# Autodesk Inventor assembly: V1
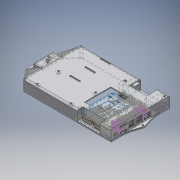
[picture p0: Inventor's stored thumbnail of the model, 180x180]
Saved by Autodesk Inventor 2019 (Build 230136000, 136)
## iProperties
Created: 2020-08-26
Part Number: V1
Document SubType Name: Assembly
Designer: infinity
Author: infinity
## Documents named in this file (4)
- C:\Users\infinity\Documents\GitHub\barc_hardware\Enclosure\XAVIER\V_2\V2.iam
- C:\Users\infinity\Documents\GitHub\barc_hardware\Enclosure\XAVIER\V_2\Enclosure_v2.ipt
- C:\Users\infinity\Documents\GitHub\barc_hardware\Dependencies\Nvidia Jetson XAVIER NX\XAVIER_SHROUDLESS.iam
- C:\Users\infinity\Documents\GitHub\barc_hardware\Dependencies\Arduino\Due\ARDUINO DUE.iam
## Components (3 placed, 3 different names)
1. Enclosure_v2:1 — Mate:1, Mate:2, Mate:3, Insert:1, Insert:2
2. XAVIER_SHROUDLESS:1 [sub-assembly] — Mate:1, Insert:1, Insert:2
3. ARDUINO DUE:1 [sub-assembly] — Mate:2, Mate:3
## Relationships (5: Mate 3, Insert 2)
- Mate:1: Enclosure_v2:1 ↔ XAVIER_SHROUDLESS:1
- Mate:2 (3 mm): Enclosure_v2:1 ↔ ARDUINO DUE:1
- Mate:3 (0.5 mm): Enclosure_v2:1 ↔ ARDUINO DUE:1
- Insert:1: Enclosure_v2:1 ↔ XAVIER_SHROUDLESS:1
- Insert:2: Enclosure_v2:1 ↔ XAVIER_SHROUDLESS:1
